# Autodesk Inventor assembly: AM14U5 Long ToughBox Mini 6in HiGrip 6wD
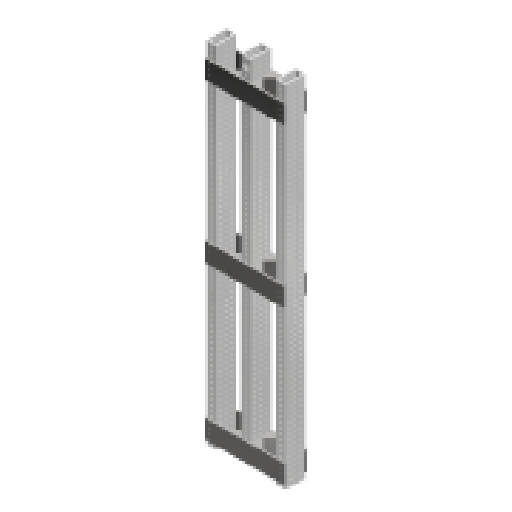
[picture p0: Inventor's stored thumbnail of the model, 512x512]
Saved by Autodesk Inventor 2027.1 (Build 311270010, 270A)
## iProperties
Created: 2023-02-01
Part Number: AM14U5 Long ToughBox Mini 6in HiGrip 6wD
Document SubType Name: Assembly
Designer: djair.oliveira
Sending System: Autodesk Translation Framework v11.17.0.187
Preprocessor: ST-DEVELOPER v19.2
Title: AM14U5 Long ToughBox Mini 6in HiGrip 6wD v5.step
## Documents named in this file (28)
- C:\Users\djair.oliveira\Documents\GitHub\MT_2026\CAD\Model C\AM14U5 Long ToughBox Mini 6in HiGrip 6wD v5\AM14U5 Long ToughBox Mini 6in HiGrip 6wD v5.iam
- C:\Users\djair.oliveira\Documents\GitHub\MT_2026\CAD\Model C\AM14U5 Long ToughBox Mini 6in HiGrip 6wD v5\AM14U5 Configurable Gearboxes_Long _TB Mini_6wD Churro Locations.iam
- C:\Users\djair.oliveira\Documents\GitHub\MT_2026\CAD\Model C\AM14U5 Long ToughBox Mini 6in HiGrip 6wD v5\375-16 x 4.25 Hex Bolt_HFBOLT 0.375-16x2.5x1-C.ipt
- C:\Users\djair.oliveira\Documents\GitHub\MT_2026\CAD\Model C\AM14U5 Long ToughBox Mini 6in HiGrip 6wD v5\2022 6 HiGrip with hub and double pulley.iam
- C:\Users\djair.oliveira\Documents\GitHub\MT_2026\CAD\Model C\AM14U5 Long ToughBox Mini 6in HiGrip 6wD v5\2022 6 HiGrip with bearings, pulleys and spacers.iam
- C:\Users\djair.oliveira\Documents\GitHub\MT_2026\CAD\Model C\AM14U5 Long ToughBox Mini 6in HiGrip 6wD v5\800-5M-15 v2.ipt
- C:\Users\djair.oliveira\Documents\GitHub\MT_2026\CAD\Model C\AM14U5 Long ToughBox Mini 6in HiGrip 6wD v5\2022 6 HiGrip with bearings, pulleys and spacers (1).iam
- C:\Users\djair.oliveira\Documents\GitHub\MT_2026\CAD\Model C\AM14U5 Long ToughBox Mini 6in HiGrip 6wD v5\375-16 Lock Nut_91831A127.ipt
- C:\Users\djair.oliveira\Documents\GitHub\MT_2026\CAD\Model C\AM14U5 Long ToughBox Mini 6in HiGrip 6wD v5\2022 6 HiGrip with bearings, pulleys and spacers (2).iam
- C:\Users\djair.oliveira\Documents\GitHub\MT_2026\CAD\Model C\AM14U5 Long ToughBox Mini 6in HiGrip 6wD v5\2022 6 HiGrip with hub and double pulley (1).iam
- C:\Users\djair.oliveira\Documents\GitHub\MT_2026\CAD\Model C\AM14U5 Long ToughBox Mini 6in HiGrip 6wD v5\2022 6 HiGrip with bearings, pulleys and spacers (3).iam
- C:\Users\djair.oliveira\Documents\GitHub\MT_2026\CAD\Model C\AM14U5 Long ToughBox Mini 6in HiGrip 6wD v5\2022 6 HiGrip with bearings, pulleys and spacers_1.iam
- C:\Users\djair.oliveira\Documents\GitHub\MT_2026\CAD\Model C\AM14U5 Long ToughBox Mini 6in HiGrip 6wD v5\2022 6 HiGrip with bearings, pulleys and spacers_2.iam
- C:\Users\djair.oliveira\Documents\GitHub\MT_2026\CAD\Model C\AM14U5 Long ToughBox Mini 6in HiGrip 6wD v5\2.iam
- C:\Users\djair.oliveira\Documents\GitHub\MT_2026\CAD\Model C\AM14U5 Long ToughBox Mini 6in HiGrip 6wD v5\2 (1).iam
- C:\Users\djair.oliveira\Documents\GitHub\MT_2026\CAD\Model C\AM14U5 Long ToughBox Mini 6in HiGrip 6wD v5\2022 6 HiGrip with bearings, pulleys and spacers_3.iam
- C:\Users\djair.oliveira\Documents\GitHub\MT_2026\CAD\Model C\AM14U5 Long ToughBox Mini 6in HiGrip 6wD v5\2022 6 HiGrip with bearings, pulleys and spacers_4.iam
- C:\Users\djair.oliveira\Documents\GitHub\MT_2026\CAD\Model C\AM14U5 Long ToughBox Mini 6in HiGrip 6wD v5\2 (1)_1.iam
- C:\Users\djair.oliveira\Documents\GitHub\MT_2026\CAD\Model C\AM14U5 Long ToughBox Mini 6in HiGrip 6wD v5\6_ Perf Wheel v3.iam
- C:\Users\djair.oliveira\Documents\GitHub\MT_2026\CAD\Model C\AM14U5 Long ToughBox Mini 6in HiGrip 6wD v5\6_ Perf Wheel v3_1.iam
- C:\Users\djair.oliveira\Documents\GitHub\MT_2026\CAD\Model C\AM14U5 Long ToughBox Mini 6in HiGrip 6wD v5\Peça118.ipt
- C:\Users\djair.oliveira\Documents\GitHub\MT_2026\CAD\Model C\Intake\Guia - Intake.ipt
- C:\Users\djair.oliveira\Documents\GitHub\MT_2026\CAD\Model C\Intake\Intake.iam
- C:\Users\djair.oliveira\Documents\GitHub\MT_2026\CAD\Model C\Elevador\Forja - Base Chassi.ipt
- C:\Users\djair.oliveira\Documents\GitHub\MT_2026\CAD\Model C\Elevador\Elevador.iam
- C:\Users\djair.oliveira\Documents\GitHub\MT_2026\CAD\Model C\Hand\Hand.iam
- C:\Users\djair.oliveira\Documents\GitHub\MT_2026\CAD\Model C\Bumper.ipt
- C:\Users\djair.oliveira\Documents\GitHub\MT_2026\CAD\Model C\Intake\Coletor - Intake.ipt
## Components (36 placed, 21 different names)
1. AM14U5 Configurable Gearboxes_Long |TB Mini|6wD Churro Locations:1 [sub-assembly] — Coincidente:1, Coincidente:2, Coincidente:3, Coincidente:4, Coincidente:5, Coincidente:6, Coincidente:9, Alinhado:1, Tangente:3, Coincidente:14, Coincidente:15, Alinhado:3
2. 375-16 x 4.25 Hex Bolt_HFBOLT 0.375-16x2.5x1-C:1
3. 2022 6 HiGrip with hub and double pulley:1 [sub-assembly]
4. 2022 6 HiGrip with bearings, pulleys and spacers:1 [sub-assembly]
5. 800-5M-15 v2:1
6. 800-5M-15 v2:2
7. 2022 6 HiGrip with bearings, pulleys and spacers (1):1 [sub-assembly]
8. 375-16 x 4.25 Hex Bolt_HFBOLT 0.375-16x2.5x1-C:2
9. 375-16 Lock Nut_91831A127:2
10. 2022 6 HiGrip with bearings, pulleys and spacers (2):1 [sub-assembly]
11. 800-5M-15 v2:3
12. 2022 6 HiGrip with hub and double pulley (1):1 [sub-assembly]
13. 2022 6 HiGrip with bearings, pulleys and spacers (3):1 [sub-assembly]
14. 375-16 x 4.25 Hex Bolt_HFBOLT 0.375-16x2.5x1-C:3
15. 375-16 Lock Nut_91831A127:3
16. 375-16 Lock Nut_91831A127:4
17. 375-16 x 4.25 Hex Bolt_HFBOLT 0.375-16x2.5x1-C:4
18. 800-5M-15 v2:4
19. 2022 6 HiGrip with bearings, pulleys and spacers:2 [sub-assembly]
20. 2022 6 HiGrip with bearings, pulleys and spacers:3 [sub-assembly]
21. 2:1 [sub-assembly]
22. 2 (1):1 [sub-assembly]
23. 2022 6 HiGrip with bearings, pulleys and spacers:4 [sub-assembly]
24. 2022 6 HiGrip with bearings, pulleys and spacers:5 [sub-assembly]
25. 2 (1):2 [sub-assembly]
26. 6" Perf Wheel v3:1 [sub-assembly]
27. 6" Perf Wheel v3:2 [sub-assembly]
28. Peça118
29. Guia - Intake:1 — Coincidente:1, Coincidente:2, Coincidente:3, Coincidente:8
30. Guia - Intake:2 — Coincidente:4, Coincidente:5, Coincidente:6, Coincidente:7, Tangente:1, Tangente:2
31. Intake:1 [sub-assembly] — Coincidente:7, Tangente:1, Tangente:2, Coincidente:8, Coincidente:16, Coincidente:17
32. Forja - Base Chassi:1 — Coincidente:9, Alinhado:1, Tangente:3, Coincidente:10, Alinhado:2, Coincidente:11
33. Elevador:1 [sub-assembly] — Coincidente:10, Alinhado:2, Coincidente:11, Coincidente:12, Coincidente:13
34. Hand:1 [sub-assembly] — Coincidente:12, Coincidente:13
35. Bumper:1 — Coincidente:14, Coincidente:15, Alinhado:3
36. Coletor - Intake:1 — Coincidente:16, Coincidente:17
## Relationships (23: Mate 17, Tangent 3, Flush 3)
- Coincidente:1 [Mate]: AM14U5 Configurable Gearboxes_Long |TB Mini|6wD Churro Locations:1 ↔ Guia - Intake:1
- Coincidente:2 [Mate]: AM14U5 Configurable Gearboxes_Long |TB Mini|6wD Churro Locations:1 ↔ Guia - Intake:1
- Coincidente:3 [Mate]: AM14U5 Configurable Gearboxes_Long |TB Mini|6wD Churro Locations:1 ↔ Guia - Intake:1
- Coincidente:4 [Mate]: AM14U5 Configurable Gearboxes_Long |TB Mini|6wD Churro Locations:1 ↔ Guia - Intake:2
- Coincidente:5 [Mate]: AM14U5 Configurable Gearboxes_Long |TB Mini|6wD Churro Locations:1 ↔ Guia - Intake:2
- Coincidente:6 [Mate]: AM14U5 Configurable Gearboxes_Long |TB Mini|6wD Churro Locations:1 ↔ Guia - Intake:2
- Coincidente:7 [Mate]: Guia - Intake:2 ↔ Intake:1
- Tangente:1: Guia - Intake:2 ↔ Intake:1
- Tangente:2: Guia - Intake:2 ↔ Intake:1
- Coincidente:8 [Mate]: Guia - Intake:1 ↔ Intake:1
- Coincidente:9 [Mate]: AM14U5 Configurable Gearboxes_Long |TB Mini|6wD Churro Locations:1 ↔ Forja - Base Chassi:1
- Alinhado:1 [Flush]: AM14U5 Configurable Gearboxes_Long |TB Mini|6wD Churro Locations:1 ↔ Forja - Base Chassi:1
- Tangente:3: AM14U5 Configurable Gearboxes_Long |TB Mini|6wD Churro Locations:1 ↔ Forja - Base Chassi:1
- Coincidente:10 [Mate]: Forja - Base Chassi:1 ↔ Elevador:1
- Alinhado:2 [Flush]: Forja - Base Chassi:1 ↔ Elevador:1
- Coincidente:11 [Mate] (-0.111 mm): Forja - Base Chassi:1 ↔ Elevador:1
- Coincidente:12 [Mate]: Elevador:1 ↔ Hand:1
- Coincidente:13 [Mate]: Elevador:1 ↔ Hand:1
- Coincidente:14 [Mate] (2 mm): AM14U5 Configurable Gearboxes_Long |TB Mini|6wD Churro Locations:1 ↔ Bumper:1
- Coincidente:15 [Mate] (2 mm): AM14U5 Configurable Gearboxes_Long |TB Mini|6wD Churro Locations:1 ↔ Bumper:1
- Alinhado:3 [Flush]: AM14U5 Configurable Gearboxes_Long |TB Mini|6wD Churro Locations:1 ↔ Bumper:1
- Coincidente:16 [Mate]: Intake:1 ↔ Coletor - Intake:1
- Coincidente:17 [Mate]: Intake:1 ↔ Coletor - Intake:1
